# Autodesk Inventor assembly: vexGripperAssembly
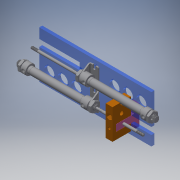
[picture p0: Inventor's stored thumbnail of the model, 180x180]
Saved by Autodesk Inventor 2016 SP1 (Build 200210100, 210)
## iProperties
Created: 2015-11-23
Part Number: vexGripperAssembly
Document SubType Name: Assembly
Designer: steele
Author: steele
## Documents named in this file (6)
- C:\snobotics\CAD-Development\robSteele\SnoBoticsSummer2015\Gripper\vexGripperAssembly.iam
- C:\snobotics\CAD-Development\robSteele\SnoBoticsSummer2015\Gripper\vexPlate.ipt
- C:\snobotics\CAD-MfgResources\McMaster-Carr\Air Cylinder\Universal Mount\Double Acting\4 in Stroke\4952K126.ipt
- C:\snobotics\CAD-MfgResources\McMaster-Carr\Air Cylinder\Universal Mount\Double Acting\3 in Stroke\6498K605.ipt
- C:\snobotics\CAD-Development\robSteele\SnoBoticsSummer2015\Gripper\vexSupportForArm.ipt
- C:\snobotics\CAD-Development\robSteele\SnoBoticsSummer2015\Gripper\vexOverSupportForArm.ipt
## Components (7 placed, 5 different names)
1. vexPlate:1 — Mate:1, Insert:1, Insert:2, Insert:3, Insert:4, Mate:2, Mate:3, Mate:6
2. 4952K126:1 — Mate:1, Insert:1, Insert:2, Insert:5
3. 4952K126:2 — Insert:3, Insert:4, Insert:6
4. 6498K605:1 — Insert:5
5. 6498K605:2 — Insert:6
6. vexSupportForArm:1 — Mate:2, Mate:3, Mate:4, Mate:5, Flush:1, Mate:6
7. vexOverSupportForArm:1 — Mate:4, Mate:5, Flush:1
## Relationships (13: Mate 6, Insert 6, Flush 1)
- Mate:1: vexPlate:1 ↔ 4952K126:1
- Insert:1: vexPlate:1 ↔ 4952K126:1
- Insert:2: vexPlate:1 ↔ 4952K126:1
- Insert:3: vexPlate:1 ↔ 4952K126:2
- Insert:4: vexPlate:1 ↔ 4952K126:2
- Insert:5: 4952K126:1 ↔ 6498K605:1
- Insert:6: 4952K126:2 ↔ 6498K605:2
- Mate:2 (0.381 mm): vexPlate:1 ↔ vexSupportForArm:1
- Mate:3: vexPlate:1 ↔ vexSupportForArm:1
- Mate:4: vexSupportForArm:1 ↔ vexOverSupportForArm:1
- Mate:5 (0.254 mm): vexSupportForArm:1 ↔ vexOverSupportForArm:1
- Flush:1: vexSupportForArm:1 ↔ vexOverSupportForArm:1
- Mate:6 (25.4 mm): vexPlate:1 ↔ vexSupportForArm:1
